# Autodesk Inventor assembly: mangOH box
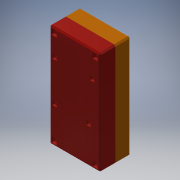
[picture p0: Inventor's stored thumbnail of the model, 180x180]
Saved by Autodesk Inventor 2017.3 (Build 213256000, 256)
## iProperties
Created: 2018-01-31
Part Number: mangOH box
Document SubType Name: Assembly
Designer: michiel
Author: michiel
## Documents named in this file (3)
- C:\Users\michiel\Documents\Inventor\mangOH box\mangOH box.iam
- C:\Users\michiel\Documents\Inventor\mangOH box\mangOH bottom.ipt
- C:\Users\michiel\Documents\Inventor\mangOH box\mangOH top.ipt
## Components (2 placed, 2 different names)
1. mangOH bottom:1 — Flush:1, Flush:2, Mate:1
2. mangOH top:1 — Flush:1, Flush:2, Mate:1
## Relationships (3: Flush 2, Mate 1)
- Flush:1: mangOH bottom:1 ↔ mangOH top:1
- Flush:2: mangOH bottom:1 ↔ mangOH top:1
- Mate:1: mangOH bottom:1 ↔ mangOH top:1
